# Autodesk Inventor assembly: proxima_sensor_model
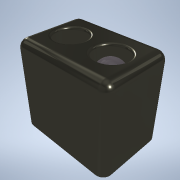
[picture p0: Inventor's stored thumbnail of the model, 180x180]
Saved by Autodesk Inventor 2021 (Build 250183000, 183)
## iProperties
Created: 2021-08-02
Part Number: proxima_sensor_model
Document SubType Name: Assembly
Designer: ermoz
Author: ermoz
## Documents named in this file (3)
- D:\Moje Wyczyny\My_Poor_Projects\Proxima_sensor\proxima-sensor\version_1.xx\proxima_sensor_case\proxima_sensor_model.iam
- D:\Moje Wyczyny\My_Poor_Projects\Proxima_sensor\proxima-sensor\version_1.xx\proxima_sensor_case\proxima_case.ipt
- D:\Moje Wyczyny\My_Poor_Projects\Proxima_sensor\proxima-sensor\version_1.xx\proxima_sensor_case\exported_from_kicad\proxima_kicadproxima_sensor_board.iam
## Components (2 placed, 2 different names)
1. proxima_case:1 — Mate:1, Mate:2, Flush:1, Angle:1
2. proxima_kicadproxima_sensor_board:1 [sub-assembly] — Mate:1, Mate:2, Flush:1, Mate:3
## Relationships (5: Mate 3, Flush 1, Angle 1)
- Mate:1 (0.1 mm): proxima_case:1 ↔ proxima_kicadproxima_sensor_board:1
- Mate:2 (0.1 mm): proxima_case:1 ↔ proxima_kicadproxima_sensor_board:1
- Flush:1 (2 mm): proxima_case:1 ↔ proxima_kicadproxima_sensor_board:1
- Mate:3: proxima_kicadproxima_sensor_board:1
- Angle:1 (0 deg): proxima_case:1
